# Autodesk Inventor assembly: ASY SLM 1210 MAIN FRAME
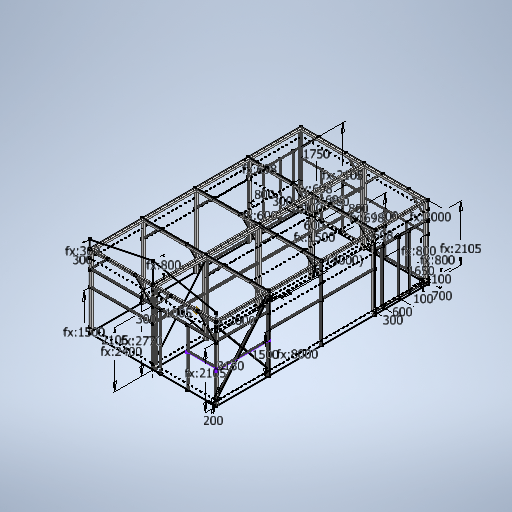
[picture p0: Inventor's stored thumbnail of the model, 512x512]
Saved by Autodesk Inventor 2025.4 (Build 294407000, 407)
## iProperties
_SolveAssemblyDoc: Frame Generator Solve Assembly
_Version: 25.0.0
Created: 2026-01-26
Part Number: ASY SLM 1210 MAIN FRAME
Document SubType Name: Assembly
Designer: admin
Mass: 845550 g
Surface Area: 739882 cm^2
Volume: 107713 cm^3
Density: 7.85 g/cm^3
Author: admin
## Documents named in this file (5)
- C:\Users\admin\Documents\Inventor\SLM-Salemal\ASY SLM 1210 MAIN FRAME.iam
- C:\Users\admin\Documents\Inventor\SLM-Salemal\PNS-1100 FRAME OLD sketch.ipt
- C:\Users\admin\Documents\Inventor\SLM-Salemal\ASY SLM 1210 MAIN FRAME\Frame\Frame 1769424024765.iam
- C:\Users\admin\Documents\Inventor\SLM-Salemal\SLM frame 4.1 D-ring.ipt
- C:\Users\admin\Documents\Inventor\SLM-Salemal\SLM frame 4.2 reinf.ipt
## Components (6 placed, 4 different names)
1. PNS-1121 FRAME OLD sketch:1 — Flush:1, Mate:1, Flush:2
2. Frame 1769424024765:1 [sub-assembly] — Mate:2, Mate:3, Mate:5, Mate:6, Flush:4
3. SLM frame 4.1 D-ring:1 — Tangent:1, Angle:1, Mate:4, Flush:3
4. SLM frame 4.2 reinf:1 — Mate:2, Mate:3, Tangent:1, Angle:1, Mate:4, Flush:3
5. SLM frame 4.2 reinf:2 — Mate:5, Mate:6, Rotational:1, Flush:4
6. SLM frame 4.1 D-ring:2 — Rotational:1
## Relationships (13: Mate 6, Flush 4, Tangent 1, Angle 1, RevoluteJoint 1)
- Flush:1: PNS-1121 FRAME OLD sketch:1
- Mate:1: PNS-1121 FRAME OLD sketch:1
- Flush:2: PNS-1121 FRAME OLD sketch:1
- Mate:2: Frame 1769424024765:1 ↔ SLM frame 4.2 reinf:1
- Mate:3: Frame 1769424024765:1 ↔ SLM frame 4.2 reinf:1
- Tangent:1: SLM frame 4.1 D-ring:1 ↔ SLM frame 4.2 reinf:1
- Angle:1 (45 deg): SLM frame 4.1 D-ring:1 ↔ SLM frame 4.2 reinf:1
- Mate:4: SLM frame 4.1 D-ring:1 ↔ SLM frame 4.2 reinf:1
- Flush:3 (10 mm): SLM frame 4.1 D-ring:1 ↔ SLM frame 4.2 reinf:1
- Mate:5: Frame 1769424024765:1 ↔ SLM frame 4.2 reinf:2
- Mate:6: Frame 1769424024765:1 ↔ SLM frame 4.2 reinf:2
- Rotational:1 [RevoluteJoint] (-10 mm): SLM frame 4.2 reinf:2 ↔ SLM frame 4.1 D-ring:2
- Flush:4 (10 mm): Frame 1769424024765:1 ↔ SLM frame 4.2 reinf:2
